# Autodesk Inventor assembly: sub-frame
Saved by Autodesk Inventor 2013 (Build 170138000, 138)
## iProperties
Created: 2013-09-17
Part Number: sub-frame
Document SubType Name: Assembly
Designer: Ian
Author: Ian
## Documents named in this file (3)
- C:\Users\Ian\Documents\Inventor\xyPartStorage\loader\sub-frame.iam
- C:\Users\Ian\Documents\Inventor\xyPartStorage\80-20 models\T-slot\1515-48.ipt
- C:\Users\Ian\Documents\Inventor\xyPartStorage\angle-90-plate.ipt
## Components (18 placed, 2 different names)
1. 1515-48:1
2. 1515-48:2
3. 1515-48:3
4. 1515-48:4
5. angle-90-plate:1
6. angle-90-plate:2
7. angle-90-plate:3
8. angle-90-plate:4
9. 1515-48:5
10. 1515-48:6
11. 1515-48:7
12. 1515-48:8
13. 1515-48:9
14. 1515-48:10
15. 1515-48:11
16. 1515-48:12
17. 1515-48:13
18. 1515-48:14
## Relationships (49: Flush 30, Mate 19)
- [Flush]: 1515-48:1 ↔ angle-90-plate:3
- [Mate]: 1515-48:1 ↔ angle-90-plate:3
- [Flush]: 1515-48:1 ↔ angle-90-plate:3
- [Mate]: 1515-48:1 ↔ 1515-48:3
- [Mate]: 1515-48:3 ↔ angle-90-plate:3
- [Flush]: 1515-48:1 ↔ 1515-48:3
- [Flush]: 1515-48:1 ↔ angle-90-plate:4
- [Flush]: 1515-48:1 ↔ angle-90-plate:4
- [Mate]: 1515-48:1 ↔ angle-90-plate:4
- [Mate]: 1515-48:1 ↔ 1515-48:2
- [Mate]: 1515-48:2 ↔ angle-90-plate:4
- [Flush]: 1515-48:1 ↔ 1515-48:2
- [Mate]: 1515-48:2 ↔ angle-90-plate:1
- [Flush]: 1515-48:2 ↔ angle-90-plate:1
- [Flush]: 1515-48:3 ↔ angle-90-plate:2
- [Mate]: 1515-48:3 ↔ angle-90-plate:2
- [Mate]: 1515-48:4 ↔ angle-90-plate:1
- [Mate]: 1515-48:2 ↔ 1515-48:4
- [Flush]: 1515-48:2 ↔ 1515-48:4
- [Flush]: 1515-48:4 ↔ angle-90-plate:1
- [Flush]: 1515-48:4 ↔ angle-90-plate:2
- [Mate]: 1515-48:3 ↔ 1515-48:7
- [Mate]: 1515-48:1 ↔ 1515-48:6
- [Mate]: 1515-48:4 ↔ 1515-48:8
- [Mate]: 1515-48:3 ↔ 1515-48:5
- [Flush]: 1515-48:4 ↔ 1515-48:7
- [Flush]: 1515-48:4 ↔ 1515-48:7
- [Flush]: 1515-48:4 ↔ 1515-48:8
- [Flush]: 1515-48:1 ↔ 1515-48:5
- [Flush]: 1515-48:4 ↔ 1515-48:8
- [Flush]: 1515-48:1 ↔ 1515-48:6
- [Mate]: 1515-48:7 ↔ 1515-48:11
- [Flush]: 1515-48:7 ↔ 1515-48:11
- [Flush]: 1515-48:7 ↔ 1515-48:11
- [Flush]: 1515-48:9 ↔ 1515-48:11
- [Mate]: 1515-48:9 ↔ 1515-48:11
- [Flush]: 1515-48:9 ↔ 1515-48:11
- [Flush]: 1515-48:9 ↔ 1515-48:12
- [Flush]: 1515-48:5 ↔ 1515-48:12
- [Flush]: 1515-48:10 ↔ 1515-48:12
- [Mate]: 1515-48:10 ↔ 1515-48:12
- [Flush]: 1515-48:10 ↔ 1515-48:12
- [Flush]: 1515-48:1 ↔ 1515-48:12
- [Flush]: 1515-48:1 ↔ 1515-48:12
- [Flush]: 1515-48:9 ↔ 1515-48:12
- [Mate]: 1515-48:3 ↔ 1515-48:14
- [Flush]: 1515-48:1 ↔ 1515-48:14
- [Mate]: 1515-48:1 ↔ 1515-48:13
- [Flush]: 1515-48:2 ↔ 1515-48:13
